# Autodesk Inventor assembly: FRC Shooter
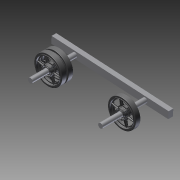
[picture p0: Inventor's stored thumbnail of the model, 180x180]
Saved by Autodesk Inventor 2012 (Build 160160000, 160)
## iProperties
Created: 2012-01-10
Part Number: FRC Shooter
Document SubType Name: Assembly
Designer: Logan
Author: Logan
## Documents named in this file (4)
- C:\Users\Logan\Desktop\FRC CAD Files\FRC Shooter.iam
- C:\Users\Logan\Desktop\FRC CAD Files\AM 6in FirstWheel\AM 6in FirstWheel.iam
- C:\Users\Logan\Desktop\FRC CAD Files\FRC Axle Base.ipt
- C:\Users\Logan\Desktop\FRC CAD Files\FRC Shooter Axle.ipt
## Components (6 placed, 3 different names)
1. AM 6in FirstWheel:1 [sub-assembly] — Mate:1, Mate:3, Angle:1, Mate:5, Rotation:2
2. AM 6in FirstWheel:2 [sub-assembly] — Mate:2, Mate:3, Mate:4, Mate:6, Mate:7, Rotation:1, Flush:3, Rotation:2
3. FRC Axle Base:1 — Insert:1, Insert:2
4. FRC Shooter Axle:1 — Insert:2, Mate:8, Flush:2
5. FRC Shooter Axle:2 — Insert:1, Mate:7, Flush:1
6. AM 6in FirstWheel:3 [sub-assembly] — Mate:8, Rotation:1, Flush:4
## Relationships (18: Mate 8, Flush 4, Angle 2, Insert 2, RelateRotation 2)
- Mate:1: AM 6in FirstWheel:1
- Mate:2: AM 6in FirstWheel:2
- Mate:3: AM 6in FirstWheel:1 ↔ AM 6in FirstWheel:2
- Mate:4: AM 6in FirstWheel:2
- Angle:1 (0 deg): AM 6in FirstWheel:1
- Mate:5: AM 6in FirstWheel:1
- Angle:2 (0 deg)
- Mate:6: AM 6in FirstWheel:2
- Insert:1: FRC Axle Base:1 ↔ FRC Shooter Axle:2
- Insert:2: FRC Axle Base:1 ↔ FRC Shooter Axle:1
- Mate:7: AM 6in FirstWheel:2 ↔ FRC Shooter Axle:2
- Mate:8: FRC Shooter Axle:1 ↔ AM 6in FirstWheel:3
- Rotation:1 [RelateRotation] (1 ul): AM 6in FirstWheel:2 ↔ AM 6in FirstWheel:3
- Flush:1 (-88.9 mm): FRC Shooter Axle:2
- Flush:2 (-107.95 mm): FRC Shooter Axle:1
- Flush:3: AM 6in FirstWheel:2
- Rotation:2 [RelateRotation] (1 ul): AM 6in FirstWheel:1 ↔ AM 6in FirstWheel:2
- Flush:4: AM 6in FirstWheel:3
